# Autodesk Inventor assembly: Assembly1
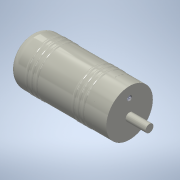
[picture p0: Inventor's stored thumbnail of the model, 180x180]
Saved by Autodesk Inventor 2022 (Build 260153000, 153)
## iProperties
Created: 2022-10-28
Part Number: Assembly1
Document SubType Name: Assembly
Designer: HP
Author: HP
## Documents named in this file (6)
- C:\CICLO IV\FUNDAMENTOS DE BIODISEÑO\BIODEÑO\Dispositivo 3.iam
- C:\CICLO IV\FUNDAMENTOS DE BIODISEÑO\BIODEÑO\Carcasa V3 Pequeño.ipt
- C:\CICLO IV\FUNDAMENTOS DE BIODISEÑO\BIODEÑO\Carcasa V3.ipt
- C:\CICLO IV\FUNDAMENTOS DE BIODISEÑO\BIODEÑO\Cella_car.ipt
- C:\CICLO IV\FUNDAMENTOS DE BIODISEÑO\BIODEÑO\BARRA V3.ipt
- C:\CICLO IV\FUNDAMENTOS DE BIODISEÑO\BIODEÑO\Tornillo 4 x 3.8.ipt
## Components (5 placed, 5 different names)
1. Carcasa V3 Pequeño:1 — Mate:1, Mate:2, Mate:11, Mate:12, Mate:13
2. Carcasa V3:1 — Mate:1, Mate:2, Mate:3, Mate:4, Mate:5, Mate:8, Mate:9
3. Cella_car:1 — Mate:3, Mate:4, Mate:5, Tangent:1
4. BARRA V3:1 — Tangent:1, Mate:13
5. Tornillo 4 x 3.8:1 — Mate:11, Mate:12
## Relationships (11: Mate 10, Tangent 1)
- Mate:1: Carcasa V3 Pequeño:1 ↔ Carcasa V3:1
- Mate:2: Carcasa V3 Pequeño:1 ↔ Carcasa V3:1
- Mate:3: Carcasa V3:1 ↔ Cella_car:1
- Mate:4: Carcasa V3:1 ↔ Cella_car:1
- Mate:5: Carcasa V3:1 ↔ Cella_car:1
- Mate:8: Carcasa V3:1
- Mate:9: Carcasa V3:1
- Mate:11: Carcasa V3 Pequeño:1 ↔ Tornillo 4 x 3.8:1
- Mate:12: Carcasa V3 Pequeño:1 ↔ Tornillo 4 x 3.8:1
- Tangent:1: Cella_car:1 ↔ BARRA V3:1
- Mate:13: Carcasa V3 Pequeño:1 ↔ BARRA V3:1
